# Autodesk Inventor assembly: RightDriveAssembly
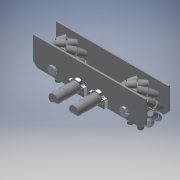
[picture p0: Inventor's stored thumbnail of the model, 180x180]
Saved by Autodesk Inventor 2017 (Build 210142000, 142)
## iProperties
Created: 2017-09-16
Part Number: RightDriveAssembly
Document SubType Name: Assembly
Designer: User
Author: User
## Documents named in this file (8)
- C:\Robotics\CAD\2017-18_CAD\RightDriveAssembly.iam
- C:\Robotics\CAD\2017-18_CAD\MecanumDriveTrainPlate17-18.ipt
- C:\Robotics\CAD\2017-18_CAD\MecanumDriveTrainPlate17-18-NoMotor.ipt
- C:\Robotics\CAD\COTSParts\Tetrix\tetrix-motor-mounts-1.snapshot.1\Tetrex 2pc motor mount.ipt
- C:\Robotics\CAD\COTSParts\Motors\Andymark 2964  NeveRest 40 Motor.ipt
- C:\Robotics\CAD\2017-18_CAD\LeftDriveTrainMecanum2017-18.iam
- C:\Robotics\CAD\COTSParts\Actobotics\615 parts\615114.ipt
- C:\Robotics\CAD\COTSParts\Actobotics\545 parts\545576.ipt
## Components (12 placed, 7 different names)
1. MecanumDriveTrainPlate17-18:1 — Insert:2, Insert:3, Insert:5
2. MecanumDriveTrainPlate17-18-NoMotor:1 — Mate:81, Mate:82, Mate:83, Mate:84
3. Tetrex 2pc motor mount:1 — Insert:2, Mate:85, Flush:1
4. Tetrex 2pc motor mount:2 — Insert:3, Mate:86, Flush:2, Insert:5
5. Andymark 2964  NeveRest 40 Motor:1 — Mate:86, Flush:2, Mate:88, Mate:89
6. Andymark 2964  NeveRest 40 Motor:2 — Mate:85, Flush:1, Mate:87, Mate:90
7. LeftDriveTrainMecanum2017-18:1 [sub-assembly] — Mate:83, Mate:84, Flush:3
8. LeftDriveTrainMecanum2017-18:2 [sub-assembly] — Mate:81, Mate:82
9. 615114:1 — Mate:87, Flush:3, Flush:4, Insert:6
10. 615114:2 — Mate:88, Flush:4, Insert:4
11. 545576:1 — Insert:6, Mate:90
12. 545576:2 — Insert:4, Mate:89
## Relationships (19: Mate 10, Insert 5, Flush 4)
- Insert:2: MecanumDriveTrainPlate17-18:1 ↔ Tetrex 2pc motor mount:1
- Insert:3: MecanumDriveTrainPlate17-18:1 ↔ Tetrex 2pc motor mount:2
- Mate:81: MecanumDriveTrainPlate17-18-NoMotor:1 ↔ LeftDriveTrainMecanum2017-18:2
- Mate:82: MecanumDriveTrainPlate17-18-NoMotor:1 ↔ LeftDriveTrainMecanum2017-18:2
- Mate:83: MecanumDriveTrainPlate17-18-NoMotor:1 ↔ LeftDriveTrainMecanum2017-18:1
- Mate:84: MecanumDriveTrainPlate17-18-NoMotor:1 ↔ LeftDriveTrainMecanum2017-18:1
- Mate:85: Tetrex 2pc motor mount:1 ↔ Andymark 2964  NeveRest 40 Motor:2
- Flush:1: Tetrex 2pc motor mount:1 ↔ Andymark 2964  NeveRest 40 Motor:2
- Mate:86: Tetrex 2pc motor mount:2 ↔ Andymark 2964  NeveRest 40 Motor:1
- Flush:2: Tetrex 2pc motor mount:2 ↔ Andymark 2964  NeveRest 40 Motor:1
- Mate:87: Andymark 2964  NeveRest 40 Motor:2 ↔ 615114:1
- Flush:3: LeftDriveTrainMecanum2017-18:1 ↔ 615114:1
- Mate:88: Andymark 2964  NeveRest 40 Motor:1 ↔ 615114:2
- Flush:4: 615114:1 ↔ 615114:2
- Insert:4: 615114:2 ↔ 545576:2
- Insert:5: MecanumDriveTrainPlate17-18:1 ↔ Tetrex 2pc motor mount:2
- Mate:89: Andymark 2964  NeveRest 40 Motor:1 ↔ 545576:2
- Insert:6: 615114:1 ↔ 545576:1
- Mate:90: Andymark 2964  NeveRest 40 Motor:2 ↔ 545576:1
